# Autodesk Inventor assembly: RobotArm
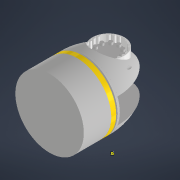
[picture p0: Inventor's stored thumbnail of the model, 180x180]
Saved by Autodesk Inventor 2021 (Build 250183000, 183)
## iProperties
Created: 2022-10-01
Part Number: RobotArm
Document SubType Name: Assembly
Designer: MicnedSQ
Author: MicnedSQ
## Documents named in this file (4)
- C:\Users\MicnedSQ\Desktop\RobotArmV1\RobotArm.iam
- C:\Users\MicnedSQ\Desktop\RobotArmV1\Base\Base.iam
- C:\Users\MicnedSQ\Desktop\RobotArmV1\RotatingBase\RotatingBase.iam
- C:\Users\MicnedSQ\Desktop\RobotArmV1\RotatingBase\CycloidalDrive\CycloidalDrive2.iam
## Components (3 placed, 3 different names)
1. Base:1 [sub-assembly] — Obrotowe:1
2. RotatingBase:1 [sub-assembly] — Obrotowe:1, Sztywne:1
3. CycloidalDrive2:1 [sub-assembly] — Sztywne:1
## Relationships (2: RevoluteJoint 1, WeldJoint 1)
- Obrotowe:1 [RevoluteJoint]: Base:1 ↔ RotatingBase:1
- Sztywne:1 [WeldJoint]: RotatingBase:1 ↔ CycloidalDrive2:1
